# Autodesk Inventor assembly: 30-00 Injectomat suplimentar
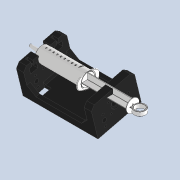
[picture p0: Inventor's stored thumbnail of the model, 180x180]
Saved by Autodesk Inventor 2020 (Build 240168000, 168)
## iProperties
Created: 2021-05-20
Part Number: 30-00 Injectomat suplimentar
Document SubType Name: Assembly
Designer: Iulian Bors
Author: Iulian Bors
## Documents named in this file (5)
- Z:\I.A.B\Proiecte\0008 I.A.B 3D 2.1 Imprimanta aracet Metal\30 Injectomat\syringe-100ml-1.snapshot.1\30-00 Injectomat suplimentar.iam
- Z:\I.A.B\Proiecte\0008 I.A.B 3D 2.1 Imprimanta aracet Metal\30 Injectomat\syringe-100ml-1.snapshot.1\Corp.ipt
- Z:\I.A.B\Proiecte\0008 I.A.B 3D 2.1 Imprimanta aracet Metal\30 Injectomat\syringe-100ml-1.snapshot.1\Cauciuc.ipt
- Z:\I.A.B\Proiecte\0008 I.A.B 3D 2.1 Imprimanta aracet Metal\30 Injectomat\syringe-100ml-1.snapshot.1\Syringe_100ml.ipt
- Z:\I.A.B\Proiecte\0008 I.A.B 3D 2.1 Imprimanta aracet Metal\30 Injectomat\0008-30-002 Corp_Injectomat1.ipt
## Components (4 placed, 4 different names)
1. Corp:2 — Mate:1, Mate:2
2. Cauciuc:1 — Insert:1, Mate:1
3. Syringe_100ml:1 — Insert:1, Angle:1
4. 0008-30-002 Corp_Injectomat1:1 — Mate:2
## Relationships (4: Mate 2, Insert 1, Angle 1)
- Insert:1: Cauciuc:1 ↔ Syringe_100ml:1
- Mate:1: Corp:2 ↔ Cauciuc:1
- Angle:1 (0 deg): Syringe_100ml:1
- Mate:2: Corp:2 ↔ 0008-30-002 Corp_Injectomat1:1
